# Autodesk Inventor assembly: WheelAssembly
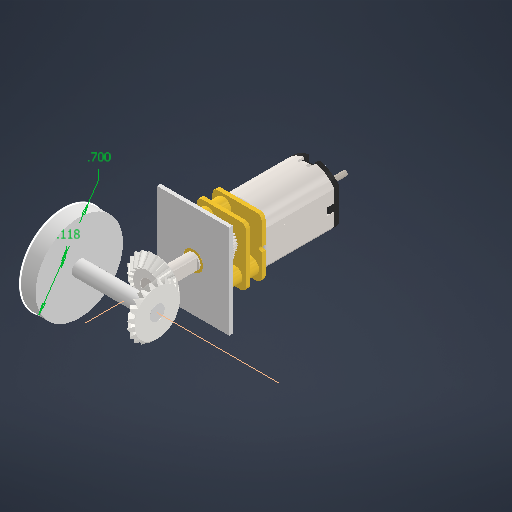
[picture p0: Inventor's stored thumbnail of the model, 512x512]
Saved by Autodesk Inventor 2026.1 (Build 301233000, 233)
## iProperties
Created: 2026-07-02
Part Number: WheelAssembly
Document SubType Name: Assembly
Designer: Kasi Pusuluri
Author: Kasi Pusuluri
## Documents named in this file (5)
- C:\Users\Kasi Pusuluri\Documents\Outpost 2026\BumperCarV2\WheelAssembly.iam
- C:\Users\Kasi Pusuluri\Documents\Outpost 2026\BumperCarV2\BumperWheel2.ipt
- C:\Users\Kasi Pusuluri\Documents\Outpost 2026\BumperCarV2\N20Motor.ipt
- C:\Users\Kasi Pusuluri\Documents\Outpost 2026\BumperCarV2\BevelGear.ipt
- C:\Users\Kasi Pusuluri\Documents\Outpost 2026\BumperCarV2\MotorProtector.ipt
## Components (5 placed, 4 different names)
1. BumperWheel2:1 — Rotational:1, Mate:1
2. N20Motor:1 — Rotational:2, Mate:2, Rotational:3
3. Bevel Gear1:1 — Rotational:1, Mate:1
4. Bevel Gear1:2 — Rotational:2, Mate:2
5. MotorProtector:1 — Rotational:3
## Relationships (5: RevoluteJoint 3, Mate 2)
- Rotational:1 [RevoluteJoint]: BumperWheel2:1 ↔ Bevel Gear1:1
- Rotational:2 [RevoluteJoint]: N20Motor:1 ↔ Bevel Gear1:2
- Mate:1: BumperWheel2:1 ↔ Bevel Gear1:1
- Mate:2: N20Motor:1 ↔ Bevel Gear1:2
- Rotational:3 [RevoluteJoint]: N20Motor:1 ↔ MotorProtector:1
